# Autodesk Inventor assembly: 部件1
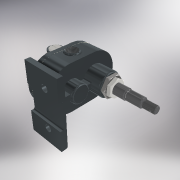
[picture p0: Inventor's stored thumbnail of the model, 180x180]
Saved by Autodesk Inventor 2020 (Build 240168000, 168)
## iProperties
Created: 2021-04-21
Part Number: 部件1
Document SubType Name: Assembly
Designer: Luorily
Author: Luorily
## Documents named in this file (15)
- E:\University\学习\工程图学\inventor上机-王静\齿轮油泵\部件1.iam
- E:\University\学习\工程图学\inventor上机-王静\齿轮油泵\泵体.ipt
- E:\University\学习\工程图学\inventor上机-王静\齿轮油泵\主动齿轮轴.ipt
- E:\University\学习\工程图学\inventor上机-王静\齿轮油泵\从动齿轮轴.ipt
- E:\University\学习\工程图学\inventor上机-王静\齿轮油泵\锁紧螺母.ipt
- E:\University\学习\工程图学\inventor上机-王静\齿轮油泵\填料压盖.ipt
- E:\University\学习\工程图学\inventor上机-王静\齿轮油泵\垫片.ipt
- E:\University\学习\工程图学\inventor上机-王静\齿轮油泵\泵盖.ipt
- C:\Users\Luorily\Documents\Inventor\Content Center Files\R2020\zh-CN\GB_T 97.1-2002\平垫圈 GB_T 97.1 6.ipt
- C:\Users\Luorily\Documents\Inventor\Content Center Files\R2020\zh-CN\GB_T 5782-2000\螺栓 GB_T 5782 M6 x 30.ipt
- C:\Users\Luorily\Documents\Inventor\Content Center Files\R2020\zh-CN\GB_T 117-2000\锥形销 GB_T 117 A 5 x 18.ipt
- C:\Users\Luorily\Desktop\学习\工程图学\inventor上机-王静\齿轮油泵\钢珠.ipt
- C:\Users\Luorily\Desktop\学习\工程图学\inventor上机-王静\齿轮油泵\钢珠定位圈.ipt
- C:\Users\Luorily\Desktop\学习\工程图学\inventor上机-王静\齿轮油泵\螺塞.ipt
- C:\Users\Luorily\Desktop\学习\工程图学\inventor上机-王静\齿轮油泵\弹簧.ipt
## Components (25 placed, 14 different names)
1. 泵体:1 — 配合:1, 配合:2, 配合:3, 配合:4, 配合:5, 配合:9, 配合:10, 配合:11, 配合:13, 配合:14, 角度:1
2. 主动齿轮轴:1 — 配合:1, 配合:3, 配合:6, 配合:7, 转动:1, 角度:1
3. 从动齿轮轴:1 — 配合:2, 配合:4, 转动:1
4. 锁紧螺母:2 — 配合:5, 配合:6, 配合:8
5. 填料压盖:1 — 配合:7, 配合:8
6. 垫片:1 — 配合:9, 配合:10, 配合:11, 配合:12
7. 泵盖:1 — 配合:12, 配合:13, 配合:14, 插入:1, 插入:2, 插入:3, 插入:4, 插入:5, 插入:6, 插入:11, 插入:13, 插入:14, 配合:15, 相切:1, 配合:16, 插入:15
8. 垫圈 GB/T 97.1-2002 6:1 — 插入:2
9. 垫圈 GB/T 97.1-2002 6:2 — 插入:6, 插入:9
10. 垫圈 GB/T 97.1-2002 6:3 — 插入:3, 插入:12
11. 垫圈 GB/T 97.1-2002 6:4 — 插入:4, 插入:7
12. 垫圈 GB/T 97.1-2002 6:5 — 插入:1, 插入:10
13. 垫圈 GB/T 97.1-2002 6:6 — 插入:5, 插入:8
14. 螺栓 GB/T 5782-2000 M6x30:1 — 插入:7
15. 螺栓 GB/T 5782-2000 M6x30:2 — 插入:8
16. 螺栓 GB/T 5782-2000 M6x30:3 — 插入:11
17. 螺栓 GB/T 5782-2000 M6x30:4 — 插入:12
18. 螺栓 GB/T 5782-2000 M6x30:5 — 插入:10
19. 螺栓 GB/T 5782-2000 M6x30:6 — 插入:9
20. 销 GB/T 117-2000 A 5 x 18:1 — 插入:14
21. 销 GB/T 117-2000 A 5 x 18:2 — 插入:13
22. 钢珠:1 — 配合:15, 相切:1, 相切:2
23. 钢珠定位圈:1 — 配合:16, 相切:2, 配合:17, 配合:18
24. 螺塞:1 — 插入:15
25. 弹簧:1 — 配合:17, 配合:18
## Relationships (37: Mate 18, Insert 15, Tangent 2, RelateRotation 1, Angle 1)
- 配合:1 [Mate]: 泵体:1 ↔ 主动齿轮轴:1
- 配合:2 [Mate]: 泵体:1 ↔ 从动齿轮轴:1
- 配合:3 [Mate]: 泵体:1 ↔ 主动齿轮轴:1
- 配合:4 [Mate]: 泵体:1 ↔ 从动齿轮轴:1
- 配合:5 [Mate]: 泵体:1 ↔ 锁紧螺母:2
- 配合:6 [Mate]: 主动齿轮轴:1 ↔ 锁紧螺母:2
- 配合:7 [Mate]: 主动齿轮轴:1 ↔ 填料压盖:1
- 配合:8 [Mate]: 锁紧螺母:2 ↔ 填料压盖:1
- 转动:1 [RelateRotation] (1 ul): 主动齿轮轴:1 ↔ 从动齿轮轴:1
- 配合:9 [Mate]: 泵体:1 ↔ 垫片:1
- 配合:10 [Mate]: 泵体:1 ↔ 垫片:1
- 配合:11 [Mate]: 泵体:1 ↔ 垫片:1
- 配合:12 [Mate]: 垫片:1 ↔ 泵盖:1
- 配合:13 [Mate]: 泵体:1 ↔ 泵盖:1
- 配合:14 [Mate]: 泵体:1 ↔ 泵盖:1
- 插入:1 [Insert]: 泵盖:1 ↔ 垫圈 GB/T 97.1-2002 6:5
- 插入:2 [Insert]: 泵盖:1 ↔ 垫圈 GB/T 97.1-2002 6:1
- 插入:3 [Insert]: 泵盖:1 ↔ 垫圈 GB/T 97.1-2002 6:3
- 插入:4 [Insert]: 泵盖:1 ↔ 垫圈 GB/T 97.1-2002 6:4
- 插入:5 [Insert]: 泵盖:1 ↔ 垫圈 GB/T 97.1-2002 6:6
- 插入:6 [Insert]: 泵盖:1 ↔ 垫圈 GB/T 97.1-2002 6:2
- 插入:7 [Insert]: 垫圈 GB/T 97.1-2002 6:4 ↔ 螺栓 GB/T 5782-2000 M6x30:1
- 插入:8 [Insert]: 垫圈 GB/T 97.1-2002 6:6 ↔ 螺栓 GB/T 5782-2000 M6x30:2
- 插入:9 [Insert]: 垫圈 GB/T 97.1-2002 6:2 ↔ 螺栓 GB/T 5782-2000 M6x30:6
- 插入:10 [Insert]: 垫圈 GB/T 97.1-2002 6:5 ↔ 螺栓 GB/T 5782-2000 M6x30:5
- 插入:11 [Insert]: 泵盖:1 ↔ 螺栓 GB/T 5782-2000 M6x30:3
- 插入:12 [Insert]: 垫圈 GB/T 97.1-2002 6:3 ↔ 螺栓 GB/T 5782-2000 M6x30:4
- 插入:13 [Insert]: 泵盖:1 ↔ 销 GB/T 117-2000 A 5 x 18:2
- 插入:14 [Insert]: 泵盖:1 ↔ 销 GB/T 117-2000 A 5 x 18:1
- 角度:1 [Angle] (799 deg): 泵体:1 ↔ 主动齿轮轴:1
- 配合:15 [Mate]: 泵盖:1 ↔ 钢珠:1
- 相切:1 [Tangent]: 泵盖:1 ↔ 钢珠:1
- 配合:16 [Mate]: 泵盖:1 ↔ 钢珠定位圈:1
- 相切:2 [Tangent]: 钢珠:1 ↔ 钢珠定位圈:1
- 插入:15 [Insert]: 泵盖:1 ↔ 螺塞:1
- 配合:17 [Mate]: 钢珠定位圈:1 ↔ 弹簧:1
- 配合:18 [Mate]: 钢珠定位圈:1 ↔ 弹簧:1
